# Autodesk Inventor assembly: plate concept
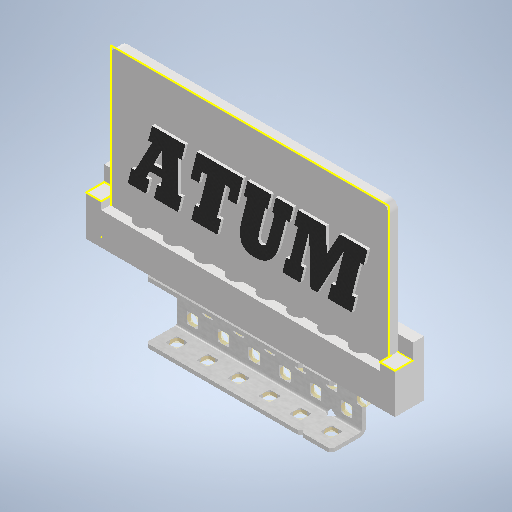
[picture p0: Inventor's stored thumbnail of the model, 512x512]
Saved by Autodesk Inventor 2025.1 (Build 291241020, 241B)
## iProperties
Created: 2024-12-05
Part Number: plate concept
Document SubType Name: Assembly
Designer: Hunter Mathis
Author: Hunter Mathis
## Documents named in this file (4)
- C:\Users\Hunter Mathis\Documents\GitHub\ATUM-V5RC-High-Stakes-CAD\Protobot\Hunter Mathis\OldVersions\plate concept.iam
- C:\Users\Hunter Mathis\Documents\GitHub\ATUM-V5RC-High-Stakes-CAD\Protobot\Hunter Mathis\plate holder.ipt
- C:\Users\Hunter Mathis\Documents\GitHub\ATUM-V5RC-High-Stakes-CAD\Protobot\Hunter Mathis\custom plate.ipt
- C:\Users\Hunter Mathis\Documents\GitHub\ATUM-V5RC-High-Stakes-CAD\VEX-CAD-Inventor\Structure\C Channel\Aluminum 1x2x1\Alu C 1x2x1x6.ipt
## Components (3 placed, 3 different names)
1. plate holder:1 — Mate:1, Mate:2, Mate:3, Mate:4, Mate:5, Mate:6
2. custom plate:1 — Mate:1, Mate:2, Mate:3
3. Alu C 1x2x1x6:1 — Mate:4, Mate:5, Mate:6
## Relationships (6: Mate 6)
- Mate:1: plate holder:1 ↔ custom plate:1
- Mate:2: plate holder:1 ↔ custom plate:1
- Mate:3: plate holder:1 ↔ custom plate:1
- Mate:4: plate holder:1 ↔ Alu C 1x2x1x6:1
- Mate:5: plate holder:1 ↔ Alu C 1x2x1x6:1
- Mate:6: plate holder:1 ↔ Alu C 1x2x1x6:1
